# Autodesk Inventor assembly: Toughbox-mini-hex-long
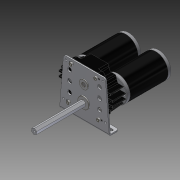
[picture p0: Inventor's stored thumbnail of the model, 180x180]
Saved by Autodesk Inventor 2014 SP1 (Build 180222100, 222)
## iProperties
Created: 2013-01-13
Part Number: Toughbox-mini-hex-long
Document SubType Name: Assembly
Designer: Moses
Mass: 3526.21 g
Surface Area: 2051.2 cm^2
Volume: 989.045 cm^3
Density: 3.56526 g/cm^3
Translation Standard: STEP AP203
FileName: S:/Products/Gearboxes Spur Single Stage/Toughbox/Toughbox Mini/Toughbox-Mini.stp
PreProcessor: Unknown
PostProcessor: Build: 138, Release: 2013 RTM - Date: Thu 03/01/2012
Sent Units: millimeter
Uncertainty: 0.001
Author: Moses
## Documents named in this file (18)
- C:\Users\Moses\Documents\Inventor\Sally Rebuild\Rebuild Sally\Toughbox-mini-hex-long.iam
- C:\Users\Moses\Documents\Inventor\Sally Rebuild\Rebuild Sally\r6zz.ipt
- C:\Users\Moses\Documents\Inventor\Sally Rebuild\Rebuild Sally\Toughbox_d07.ipt
- C:\Users\Moses\Documents\Inventor\Sally Rebuild\Rebuild Sally\Toughbox_d05.ipt
- C:\Users\Moses\Documents\Inventor\Sally Rebuild\Rebuild Sally\Toughbox_d08.ipt
- C:\Users\Moses\Documents\Inventor\Sally Rebuild\Rebuild Sally\Toughbox_d06.ipt
- C:\Users\Moses\Documents\Inventor\Sally Rebuild\Rebuild Sally\fr-6-zz.ipt
- C:\Users\Moses\Documents\Inventor\Sally Rebuild\Rebuild Sally\10-32_nylock_nut.ipt
- C:\Users\Moses\Documents\Inventor\Sally Rebuild\Rebuild Sally\5-16_washer.ipt
- C:\Users\Moses\Documents\Inventor\Sally Rebuild\Rebuild Sally\Toughbox_d09.ipt
- C:\Users\Moses\Documents\Inventor\Sally Rebuild\Rebuild Sally\8mm_spring_clip.ipt
- C:\Users\Moses\Documents\Inventor\Sally Rebuild\Rebuild Sally\Toughbox-mini_d01-5-12.ipt
- C:\Users\Moses\Documents\Inventor\Sally Rebuild\Rebuild Sally\Toughbox-mini_d02.ipt
- C:\Users\Moses\Documents\Inventor\Sally Rebuild\Rebuild Sally\10-32x0625_shcs.ipt
- C:\Users\Moses\Documents\Inventor\Sally Rebuild\Rebuild Sally\CIM motor1.ipt
- C:\Users\Moses\Documents\Inventor\Sally Rebuild\Rebuild Sally\Toughbox_d31.ipt
- C:\Users\Moses\Documents\Inventor\Sally Rebuild\Rebuild Sally\fr8zz-hex.ipt
- C:\Users\Moses\Documents\Inventor\Sally Rebuild\Rebuild Sally\97431A350.ipt
## Components (34 placed, 17 different names)
1. r6zz:1 — Mate:36, Mate:37
2. r6zz:2 — Mate:2, Mate:1, Mate:7
3. Toughbox_d31:1 — Mate:1, Mate:2, Mate:3, Mate:4, Mate:5, Mate:6, Mate:9, Mate:10, Mate:11
4. Toughbox_d07:1 — Mate:28, Mate:29, Mate:30, Mate:32, Mate:33, Mate:34, Flush:1, Flush:2, Mate:35, Mate:36, Mate:37, Rotation:4
5. Toughbox_d05:1 — Mate:31, Mate:32, Mate:33, Mate:34, Flush:1, Rotation:1, Rotation:2, Rotation:4
6. Toughbox_d08:1 — Mate:28, Mate:29, Mate:30, Mate:31
7. Toughbox_d06:1 — Mate:8, Mate:9, Mate:10, Mate:11
8. fr-6-zz:1 — Insert:10, Flush:2, Mate:35
9. fr8zz-hex:1 — Insert:3, Mate:3, Mate:4
10. 10-32_nylock_nut:1 — Mate:38, Mate:39
11. 10-32_nylock_nut:2 — Mate:40, Mate:41
12. 10-32_nylock_nut:3 — Insert:9
13. 10-32_nylock_nut:4 — Insert:8
14. 5-16_washer:1 — Mate:12, Mate:14, Mate:15
15. 5-16_washer:2 — Mate:13, Mate:15, Mate:26
16. 5-16_washer:3 — Mate:16, Mate:19, Mate:21
17. 5-16_washer:4 — Mate:17, Mate:18, Mate:19
18. Toughbox_d09:1 — Mate:25, Mate:26, Mate:27, Rotation:2
19. Toughbox_d09:2 — Mate:20, Mate:21, Mate:23, Rotation:1
20. 8mm_spring_clip:1 — Mate:24, Mate:27
21. 8mm_spring_clip:2 — Mate:22, Mate:23
22. Toughbox-mini_d01-5-12:1 — Insert:1, Insert:2, Insert:8, Insert:9, Mate:7, Mate:39, Mate:41, Insert:11, Insert:12, Insert:13, Insert:14
23. Toughbox-mini_d02:1 — Insert:3, Insert:4, Insert:5, Insert:6, Insert:7, Insert:10
24. 10-32x0625_shcs:1 — Insert:12
25. 10-32x0625_shcs:2 — Insert:5
26. 10-32x0625_shcs:3 — Insert:6, Mate:40
27. 10-32x0625_shcs:4 — Insert:7, Mate:38
28. 10-32x0625_shcs:5 — Insert:4
29. 10-32x0625_shcs:6 — Insert:11
30. 10-32x0625_shcs:7 — Insert:13
31. 10-32x0625_shcs:8 — Insert:14
32. CIM motor1:1 — Insert:1, Mate:16, Mate:17, Mate:18, Mate:20, Mate:22
33. CIM motor1:2 — Insert:2, Mate:12, Mate:13, Mate:14, Mate:24, Mate:25
34. 97431A350:1 — Mate:5, Mate:6, Mate:8
## Relationships (60: Mate 41, Insert 14, RelateRotation 3, Flush 2)
- Insert:1: Toughbox-mini_d01-5-12:1 ↔ CIM motor1:1
- Insert:2: Toughbox-mini_d01-5-12:1 ↔ CIM motor1:2
- Mate:1: r6zz:2 ↔ Toughbox_d31:1
- Mate:2: r6zz:2 ↔ Toughbox_d31:1
- Insert:3: fr8zz-hex:1 ↔ Toughbox-mini_d02:1
- Insert:4: Toughbox-mini_d02:1 ↔ 10-32x0625_shcs:5
- Insert:5: Toughbox-mini_d02:1 ↔ 10-32x0625_shcs:2
- Insert:6: Toughbox-mini_d02:1 ↔ 10-32x0625_shcs:3
- Insert:7: Toughbox-mini_d02:1 ↔ 10-32x0625_shcs:4
- Insert:8: 10-32_nylock_nut:4 ↔ Toughbox-mini_d01-5-12:1
- Insert:9: 10-32_nylock_nut:3 ↔ Toughbox-mini_d01-5-12:1
- Mate:3: Toughbox_d31:1 ↔ fr8zz-hex:1
- Mate:4: Toughbox_d31:1 ↔ fr8zz-hex:1
- Mate:5: Toughbox_d31:1 ↔ 97431A350:1
- Mate:6: Toughbox_d31:1 ↔ 97431A350:1
- Mate:7: r6zz:2 ↔ Toughbox-mini_d01-5-12:1
- Mate:8: Toughbox_d06:1 ↔ 97431A350:1
- Mate:9: Toughbox_d31:1 ↔ Toughbox_d06:1
- Mate:10: Toughbox_d31:1 ↔ Toughbox_d06:1
- Mate:11: Toughbox_d31:1 ↔ Toughbox_d06:1
- Insert:10: fr-6-zz:1 ↔ Toughbox-mini_d02:1
- Mate:12: 5-16_washer:1 ↔ CIM motor1:2
- Mate:13: 5-16_washer:2 ↔ CIM motor1:2
- Mate:14: 5-16_washer:1 ↔ CIM motor1:2
- Mate:15: 5-16_washer:1 ↔ 5-16_washer:2
- Mate:16: 5-16_washer:3 ↔ CIM motor1:1
- Mate:17: 5-16_washer:4 ↔ CIM motor1:1
- Mate:18: 5-16_washer:4 ↔ CIM motor1:1
- Mate:19: 5-16_washer:3 ↔ 5-16_washer:4
- Mate:20: Toughbox_d09:2 ↔ CIM motor1:1
- Mate:21: 5-16_washer:3 ↔ Toughbox_d09:2
- Mate:22: 8mm_spring_clip:2 ↔ CIM motor1:1
- Mate:23: Toughbox_d09:2 ↔ 8mm_spring_clip:2
- Mate:24: 8mm_spring_clip:1 ↔ CIM motor1:2
- Mate:25: Toughbox_d09:1 ↔ CIM motor1:2
- Mate:26: 5-16_washer:2 ↔ Toughbox_d09:1
- Mate:27: Toughbox_d09:1 ↔ 8mm_spring_clip:1
- Mate:28: Toughbox_d07:1 ↔ Toughbox_d08:1
- Mate:29: Toughbox_d07:1 ↔ Toughbox_d08:1
- Mate:30: Toughbox_d07:1 ↔ Toughbox_d08:1
- Mate:31: Toughbox_d05:1 ↔ Toughbox_d08:1
- Mate:32: Toughbox_d07:1 ↔ Toughbox_d05:1
- Mate:33: Toughbox_d07:1 ↔ Toughbox_d05:1
- Mate:34: Toughbox_d07:1 ↔ Toughbox_d05:1
- Flush:1: Toughbox_d07:1 ↔ Toughbox_d05:1
- Flush:2 (0.9398 mm): Toughbox_d07:1 ↔ fr-6-zz:1
- Mate:35: Toughbox_d07:1 ↔ fr-6-zz:1
- Mate:36: r6zz:1 ↔ Toughbox_d07:1
- Mate:37: r6zz:1 ↔ Toughbox_d07:1
- Mate:38: 10-32_nylock_nut:1 ↔ 10-32x0625_shcs:4
- Mate:39: 10-32_nylock_nut:1 ↔ Toughbox-mini_d01-5-12:1
- Mate:40: 10-32_nylock_nut:2 ↔ 10-32x0625_shcs:3
- Mate:41: 10-32_nylock_nut:2 ↔ Toughbox-mini_d01-5-12:1
- Insert:11: Toughbox-mini_d01-5-12:1 ↔ 10-32x0625_shcs:6
- Insert:12: Toughbox-mini_d01-5-12:1 ↔ 10-32x0625_shcs:1
- Insert:13: Toughbox-mini_d01-5-12:1 ↔ 10-32x0625_shcs:7
- Insert:14: Toughbox-mini_d01-5-12:1 ↔ 10-32x0625_shcs:8
- Rotation:1 [RelateRotation] (0.28 ul): Toughbox_d05:1 ↔ Toughbox_d09:2
- Rotation:2 [RelateRotation] (0.28 ul): Toughbox_d05:1 ↔ Toughbox_d09:1
- Rotation:4 [RelateRotation] (1 ul): Toughbox_d07:1 ↔ Toughbox_d05:1
